# Autodesk Inventor assembly: Layer2_Top_Quarter
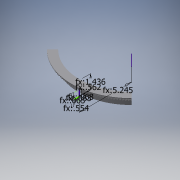
[picture p0: Inventor's stored thumbnail of the model, 180x180]
Saved by Autodesk Inventor 2017 (Build 210142000, 142)
## iProperties
Created: 2017-02-10
Part Number: Layer2_Top_Quarter
Document SubType Name: Assembly
Designer: David Kopala
Author: David Kopala
## Documents named in this file (3)
- Z:\Documents\Drone\Drone\3D Models\Project\Chassis_04\PrinterStaging\Layer2_Top_Quarter.iam
- Z:\Documents\Drone\Drone\3D Models\Project\Chassis_04\PrinterStaging\Layer2_Top_Quarter.ipt
- Z:\Documents\Drone\Drone\3D Models\Project\Chassis_04\PrinterStaging\Spur Gear11_Prep.ipt
## Components (2 placed, 2 different names)
1. Layer2_Top_Quarter:1 — Mate:1, Insert:1, Flush:1
2. Spur Gear1:1 — Mate:1, Insert:1, Flush:1
## Relationships (3: Mate 1, Insert 1, Flush 1)
- Mate:1: Layer2_Top_Quarter:1 ↔ Spur Gear1:1
- Insert:1: Layer2_Top_Quarter:1 ↔ Spur Gear1:1
- Flush:1: Layer2_Top_Quarter:1 ↔ Spur Gear1:1
